# Autodesk Inventor assembly: motor
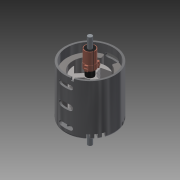
[picture p0: Inventor's stored thumbnail of the model, 180x180]
Saved by Autodesk Inventor 2018 (Build 220112000, 112)
## iProperties
Created: 2013-03-24
Part Number: motor
Material: 一般
Document SubType Name: Assembly
Designer: ku_sk
Author: ku_sk
## Documents named in this file (5)
- E:\windows\Documents\Inventor\Content Center Files\bay shooter\reedy_540_rc_motor-1.snapshot.2\inner.iam
- E:\windows\Documents\Inventor\Content Center Files\bay shooter\reedy_540_rc_motor-1.snapshot.2\motor_can.ipt
- E:\windows\Documents\Inventor\Content Center Files\bay shooter\reedy_540_rc_motor-1.snapshot.2\motor arm.iam
- E:\windows\Documents\Inventor\Content Center Files\bay shooter\reedy_540_rc_motor-1.snapshot.2\motor bushing.ipt
- E:\windows\Documents\Inventor\Content Center Files\bay shooter\reedy_540_rc_motor-1.snapshot.2\magnets.ipt
## Components (4 placed, 4 different names)
1. motor_can:1
2. motor arm:1 [sub-assembly] — メイト:1, メイト:2
3. motor bushing:2 — メイト:1, メイト:2
4. magnets:1
## Relationships (2: Mate 2)
- メイト:1 [Mate]: motor arm:1 ↔ motor bushing:2
- メイト:2 [Mate]: motor arm:1 ↔ motor bushing:2
